# Autodesk Inventor assembly: Panatogrape
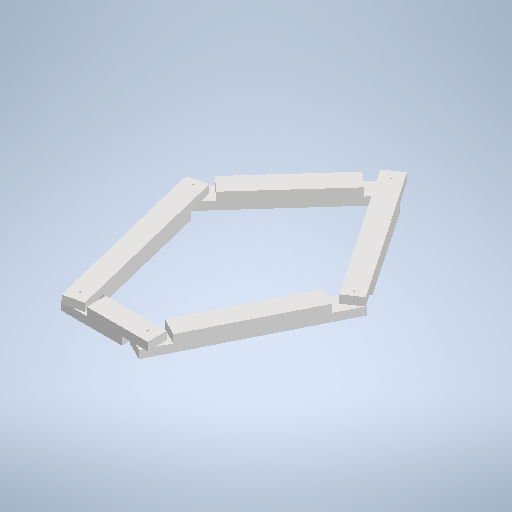
[picture p0: Inventor's stored thumbnail of the model, 512x512]
Saved by Autodesk Inventor 2025.2 (Build 292293000, 293)
## iProperties
Created: 2025-03-03
Part Number: Panatogrape
Document SubType Name: Assembly
Designer: Elisabete
Author: Elisabete
## Documents named in this file (4)
- C:\Users\Elisabete\Desktop\Ecole\Année3\Sys asservi 3\5-Bar-Parallel-Robot-via-MATLAB-Simscape-main\5-Bar-Parallel-Robot-via-MATLAB-Simscape-main\Panatogrape.iam
- C:\Users\Elisabete\Desktop\Ecole\Année3\Sys asservi 3\5-Bar-Parallel-Robot-via-MATLAB-Simscape-main\5-Bar-Parallel-Robot-via-MATLAB-Simscape-main\entremoteur.ipt
- C:\Users\Elisabete\Desktop\Ecole\Année3\Sys asservi 3\5-Bar-Parallel-Robot-via-MATLAB-Simscape-main\5-Bar-Parallel-Robot-via-MATLAB-Simscape-main\Bras_arrierre.ipt
- C:\Users\Elisabete\Desktop\Ecole\Année3\Sys asservi 3\5-Bar-Parallel-Robot-via-MATLAB-Simscape-main\5-Bar-Parallel-Robot-via-MATLAB-Simscape-main\Bras_avant.ipt
## Components (5 placed, 3 different names)
1. entremoteur:1 — Placage:1, Placage:2, Placage:3, Placage:4
2. Bras_arrierre:1 — Placage:1, Placage:2, Placage:7, Placage:8
3. Bras_arrierre:2 — Placage:3, Placage:4, Placage:5, Placage:6
4. Bras_avant:1 — Placage:5, Placage:6, Placage:9, Placage:10
5. Bras_avant:2 — Placage:7, Placage:8, Placage:9, Placage:10
## Relationships (10: Mate 10)
- Placage:1 [Mate]: entremoteur:1 ↔ Bras_arrierre:1
- Placage:2 [Mate]: entremoteur:1 ↔ Bras_arrierre:1
- Placage:3 [Mate]: entremoteur:1 ↔ Bras_arrierre:2
- Placage:4 [Mate]: entremoteur:1 ↔ Bras_arrierre:2
- Placage:5 [Mate]: Bras_arrierre:2 ↔ Bras_avant:1
- Placage:6 [Mate]: Bras_arrierre:2 ↔ Bras_avant:1
- Placage:7 [Mate]: Bras_arrierre:1 ↔ Bras_avant:2
- Placage:8 [Mate]: Bras_arrierre:1 ↔ Bras_avant:2
- Placage:9 [Mate]: Bras_avant:1 ↔ Bras_avant:2
- Placage:10 [Mate]: Bras_avant:1 ↔ Bras_avant:2
